# Autodesk Inventor assembly: Assembly1
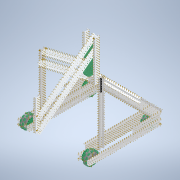
[picture p0: Inventor's stored thumbnail of the model, 180x180]
Saved by Autodesk Inventor 2020 (Build 240168000, 168)
## iProperties
Created: 2019-10-29
Part Number: Assembly1
Document SubType Name: Assembly
Designer: Alex Zaccardelli
Author: Alex Zaccardelli
## Documents named in this file (19)
- D:\DR4BTrayBot\Assembly1.iam
- D:\DR4BTrayBot\SIGBotsCADLibrary-20191023T040826Z-001\SIGBotsCADLibrary\SIGBotsCADLibrary\Structure\C-Channel 5 x 35 (aluminum).ipt
- D:\DR4BTrayBot\SIGBotsCADLibrary-20191023T040826Z-001\SIGBotsCADLibrary\SIGBotsCADLibrary\Structure\C-Channel 3 x 13 (aluminum).ipt
- D:\DR4BTrayBot\SIGBotsCADLibrary-20191023T040826Z-001\SIGBotsCADLibrary\SIGBotsCADLibrary\Structure\C-Channel 2 x 35 (aluminum) New.ipt
- D:\DR4BTrayBot\SIGBotsCADLibrary-20191023T040826Z-001\SIGBotsCADLibrary\SIGBotsCADLibrary\Motion\Spacer 0.50 unit.ipt
- D:\DR4BTrayBot\SIGBotsCADLibrary-20191023T040826Z-001\SIGBotsCADLibrary\SIGBotsCADLibrary\3_25_Omni-Directional_Wheel_276-3526.iam
- D:\DR4BTrayBot\SIGBotsCADLibrary-20191023T040826Z-001\SIGBotsCADLibrary\SIGBotsCADLibrary\Motion\Spacer 0.75 unit.ipt
- D:\DR4BTrayBot\SIGBotsCADLibrary-20191023T040826Z-001\SIGBotsCADLibrary\SIGBotsCADLibrary\Motion\Insert HS Metal.ipt
- D:\DR4BTrayBot\SIGBotsCADLibrary-20191023T040826Z-001\SIGBotsCADLibrary\SIGBotsCADLibrary\Motion\Sprocket HS 18 tooth.ipt
- D:\DR4BTrayBot\SIGBotsCADLibrary-20191023T040826Z-001\SIGBotsCADLibrary\SIGBotsCADLibrary\Structure\C-Channel 3 x 32 (aluminum).ipt
- D:\DR4BTrayBot\SIGBotsCADLibrary-20191023T040826Z-001\SIGBotsCADLibrary\SIGBotsCADLibrary\Structure\C-Channel 2 x 30 (aluminum).ipt
- D:\DR4BTrayBot\SIGBotsCADLibrary-20191023T040826Z-001\SIGBotsCADLibrary\SIGBotsCADLibrary\Motion\Bearing Block.ipt
- D:\DR4BTrayBot\SIGBotsCADLibrary-20191023T040826Z-001\SIGBotsCADLibrary\SIGBotsCADLibrary\Motion\Spacer 0.25 unit.ipt
- D:\DR4BTrayBot\SIGBotsCADLibrary-20191023T040826Z-001\SIGBotsCADLibrary\SIGBotsCADLibrary\Structure\C-Channel 2 x 20 (aluminum).ipt
- D:\DR4BTrayBot\SIGBotsCADLibrary-20191023T040826Z-001\SIGBotsCADLibrary\SIGBotsCADLibrary\Structure\C-Channel 2 x 24 (aluminum).ipt
- D:\DR4BTrayBot\SIGBotsCADLibrary-20191023T040826Z-001\SIGBotsCADLibrary\SIGBotsCADLibrary\Motion\Gear HS 84 tooth.ipt
- D:\DR4BTrayBot\SIGBotsCADLibrary-20191023T040826Z-001\SIGBotsCADLibrary\SIGBotsCADLibrary\Motion\Gear HS 12 tooth.ipt
- D:\DR4BTrayBot\SIGBotsCADLibrary-20191023T040826Z-001\SIGBotsCADLibrary\SIGBotsCADLibrary\Structure\Standoff 1.0 inch.ipt
- D:\DR4BTrayBot\SIGBotsCADLibrary-20191023T040826Z-001\SIGBotsCADLibrary\SIGBotsCADLibrary\Structure\C-Channel 2 x 15 (aluminum).ipt
## Components (56 placed, 18 different names)
1. C-Channel 5 x 35 (aluminum):1 — Mate:1, Mate:2, Mate:3, Mate:42, Mate:48, Mate:49, Mate:50, Mate:54, Mate:55, Mate:56, Mate:88, Mate:89
2. C-Channel 3 x 13 (aluminum):1 — Mate:1, Mate:2, Mate:3, Mate:7, Mate:8, Mate:9, Mate:131
3. C-Channel 2 x 35 (aluminum) New:1 — Mate:7, Mate:8, Mate:9, Mate:39, Mate:40, Mate:41, Mate:131
4. C-Channel 2 x 35 (aluminum) New:2 — Mate:25, Mate:26, Mate:45, Mate:90, Mate:152, Mate:153
5. Spacer 0.50 unit:1 — Mate:41
6. 3_25_Omni-Directional_Wheel_276-3526:1 [sub-assembly]
7. Spacer 0.75 unit:1
8. Insert HS Metal:1
9. Insert HS Metal:2
10. Sprocket HS 18 tooth:1 — Mate:25, Mate:26
11. Spacer 0.50 unit:2
12. 3_25_Omni-Directional_Wheel_276-3526:2 [sub-assembly]
13. Spacer 0.75 unit:2
14. Insert HS Metal:3
15. Insert HS Metal:4
16. Sprocket HS 18 tooth:2 — Mate:39, Mate:40
17. C-Channel 3 x 32 (aluminum):1 — Mate:42, Mate:45, Mate:88, Mate:89, Mate:90, Mate:91
18. C-Channel 3 x 13 (aluminum):2 — Mate:48, Mate:49, Mate:50, Mate:51, Mate:52, Mate:53
19. C-Channel 2 x 35 (aluminum) New:3 — Mate:51, Mate:52, Mate:53, Mate:86
20. C-Channel 3 x 32 (aluminum):2 — Mate:54, Mate:55, Mate:56, Mate:57, Mate:58, Mate:59, Mate:94
21. C-Channel 2 x 35 (aluminum) New:4 — Mate:57, Mate:58, Mate:59, Mate:72, Mate:73, Mate:87, Mate:95, Mate:96
22. Spacer 0.50 unit:3 — Mate:73
23. 3_25_Omni-Directional_Wheel_276-3526:3 [sub-assembly]
24. Spacer 0.75 unit:3
25. Insert HS Metal:5
26. Insert HS Metal:6
27. Sprocket HS 18 tooth:3 — Mate:72
28. Spacer 0.50 unit:4 — Mate:87
29. 3_25_Omni-Directional_Wheel_276-3526:4 [sub-assembly]
30. Spacer 0.75 unit:4
31. Insert HS Metal:7
32. Insert HS Metal:8
33. Sprocket HS 18 tooth:4 — Mate:86
34. C-Channel 2 x 30 (aluminum):1 — Mate:91, Mate:103, Mate:104, Mate:105, Mate:106, Mate:107, Mate:108, Mate:109, Mate:110, Mate:111, Mate:112, Mate:152, Mate:153
35. C-Channel 2 x 30 (aluminum):2 — Mate:94, Mate:95, Mate:96, Mate:97, Mate:98, Mate:99, Mate:100, Mate:101, Mate:102, Mate:113, Mate:114, Mate:115
36. Bearing Block:1 — Mate:97, Mate:98, Mate:99
37. Bearing Block:2 — Mate:100, Mate:101, Mate:102
38. Bearing Block:3 — Mate:103, Mate:104, Mate:105
39. Bearing Block:4 — Mate:106, Mate:107, Mate:108
40. C-Channel 2 x 30 (aluminum):3 — Mate:116, Mate:117, Mate:133, Mate:135, Mate:136, Flush:5, Angle:1, Mate:154
41. Spacer 0.25 unit:1 — Mate:109, Mate:110, Mate:116, Mate:117
42. Spacer 0.25 unit:2 — Mate:111, Mate:112, Mate:143
43. Spacer 0.25 unit:3 — Mate:113
44. Spacer 0.25 unit:4 — Mate:114, Mate:115
45. C-Channel 2 x 20 (aluminum):1 — Mate:133, Mate:135, Mate:137, Mate:138, Mate:139, Mate:144, Mate:145, Mate:146, Mate:147, Mate:148, Flush:7
46. Gear HS 84 tooth:1 — Mate:136, Mate:137, Flush:2, Mate:154
47. Gear HS 84 tooth:2 — Flush:2, Mate:138, Flush:3, Mate:158, Mate:159
48. Gear HS 12 tooth:1 — Mate:139, Flush:3
49. C-Channel 2 x 30 (aluminum):4 — Mate:143, Flush:5, Angle:1, Mate:144
50. C-Channel 2 x 24 (aluminum):1 — Mate:149, Mate:150, Mate:151, Mate:160, Mate:161
51. Standoff 1.0 inch:1 — Mate:145, Mate:146, Mate:149, Mate:151
52. Standoff 1.0 inch:2 — Mate:147, Mate:148, Mate:150
53. C-Channel 2 x 35 (aluminum) New:5 — Mate:158, Mate:159, Flush:6, Angle:2, Mate:164
54. C-Channel 2 x 35 (aluminum) New:6 — Flush:6, Angle:2, Mate:162, Mate:163, Mate:165
55. C-Channel 2 x 20 (aluminum):2 — Flush:7, Mate:160, Mate:161, Mate:162
56. C-Channel 2 x 15 (aluminum):1 — Mate:163, Mate:164, Mate:165
## Relationships (139: Mate 132, Flush 5, Angle 2)
- Mate:1: C-Channel 5 x 35 (aluminum):1 ↔ C-Channel 3 x 13 (aluminum):1
- Mate:2: C-Channel 5 x 35 (aluminum):1 ↔ C-Channel 3 x 13 (aluminum):1
- Mate:3: C-Channel 5 x 35 (aluminum):1 ↔ C-Channel 3 x 13 (aluminum):1
- Mate:7: C-Channel 3 x 13 (aluminum):1 ↔ C-Channel 2 x 35 (aluminum) New:1
- Mate:8: C-Channel 3 x 13 (aluminum):1 ↔ C-Channel 2 x 35 (aluminum) New:1
- Mate:9: C-Channel 3 x 13 (aluminum):1 ↔ C-Channel 2 x 35 (aluminum) New:1
- [Mate]: Spacer 0.75 unit:1 ↔ Sprocket HS 18 tooth:1
- [Mate]: Spacer 0.75 unit:1 ↔ Sprocket HS 18 tooth:1
- [Mate]: 3_25_Omni-Directional_Wheel_276-3526:1 ↔ Insert HS Metal:1
- [Mate]: 3_25_Omni-Directional_Wheel_276-3526:1 ↔ Insert HS Metal:1
- [Mate]: 3_25_Omni-Directional_Wheel_276-3526:1 ↔ Insert HS Metal:1
- [Mate]: 3_25_Omni-Directional_Wheel_276-3526:1 ↔ Insert HS Metal:2
- [Mate]: 3_25_Omni-Directional_Wheel_276-3526:1 ↔ Insert HS Metal:2
- [Mate]: 3_25_Omni-Directional_Wheel_276-3526:1 ↔ Insert HS Metal:2
- [Mate]: Spacer 0.75 unit:1 ↔ Insert HS Metal:1
- [Mate]: Spacer 0.75 unit:1 ↔ Insert HS Metal:1
- [Mate]: Spacer 0.50 unit:1 ↔ Insert HS Metal:2
- [Mate]: Spacer 0.50 unit:1 ↔ Insert HS Metal:2
- Mate:25: C-Channel 2 x 35 (aluminum) New:2 ↔ Sprocket HS 18 tooth:1
- Mate:26: C-Channel 2 x 35 (aluminum) New:2 ↔ Sprocket HS 18 tooth:1
- [Mate]: Spacer 0.75 unit:2 ↔ Sprocket HS 18 tooth:2
- [Mate]: Spacer 0.75 unit:2 ↔ Sprocket HS 18 tooth:2
- [Mate]: 3_25_Omni-Directional_Wheel_276-3526:2 ↔ Insert HS Metal:3
- [Mate]: 3_25_Omni-Directional_Wheel_276-3526:2 ↔ Insert HS Metal:3
- [Mate]: 3_25_Omni-Directional_Wheel_276-3526:2 ↔ Insert HS Metal:3
- [Mate]: 3_25_Omni-Directional_Wheel_276-3526:2 ↔ Insert HS Metal:4
- [Mate]: 3_25_Omni-Directional_Wheel_276-3526:2 ↔ Insert HS Metal:4
- [Mate]: 3_25_Omni-Directional_Wheel_276-3526:2 ↔ Insert HS Metal:4
- [Mate]: Spacer 0.75 unit:2 ↔ Insert HS Metal:3
- [Mate]: Spacer 0.75 unit:2 ↔ Insert HS Metal:3
- [Mate]: Spacer 0.50 unit:2 ↔ Insert HS Metal:4
- [Mate]: Spacer 0.50 unit:2 ↔ Insert HS Metal:4
- Mate:39: C-Channel 2 x 35 (aluminum) New:1 ↔ Sprocket HS 18 tooth:2
- Mate:40: C-Channel 2 x 35 (aluminum) New:1 ↔ Sprocket HS 18 tooth:2
- Mate:41: C-Channel 2 x 35 (aluminum) New:1 ↔ Spacer 0.50 unit:1
- Mate:42: C-Channel 5 x 35 (aluminum):1 ↔ C-Channel 3 x 32 (aluminum):1
- Mate:45: C-Channel 2 x 35 (aluminum) New:2 ↔ C-Channel 3 x 32 (aluminum):1
- Mate:48: C-Channel 5 x 35 (aluminum):1 ↔ C-Channel 3 x 13 (aluminum):2
- Mate:49: C-Channel 5 x 35 (aluminum):1 ↔ C-Channel 3 x 13 (aluminum):2
- Mate:50: C-Channel 5 x 35 (aluminum):1 ↔ C-Channel 3 x 13 (aluminum):2
- Mate:51: C-Channel 3 x 13 (aluminum):2 ↔ C-Channel 2 x 35 (aluminum) New:3
- Mate:52: C-Channel 3 x 13 (aluminum):2 ↔ C-Channel 2 x 35 (aluminum) New:3
- Mate:53: C-Channel 3 x 13 (aluminum):2 ↔ C-Channel 2 x 35 (aluminum) New:3
- Mate:54: C-Channel 5 x 35 (aluminum):1 ↔ C-Channel 3 x 32 (aluminum):2
- Mate:55: C-Channel 5 x 35 (aluminum):1 ↔ C-Channel 3 x 32 (aluminum):2
- Mate:56: C-Channel 5 x 35 (aluminum):1 ↔ C-Channel 3 x 32 (aluminum):2
- Mate:57: C-Channel 3 x 32 (aluminum):2 ↔ C-Channel 2 x 35 (aluminum) New:4
- Mate:58: C-Channel 3 x 32 (aluminum):2 ↔ C-Channel 2 x 35 (aluminum) New:4
- Mate:59: C-Channel 3 x 32 (aluminum):2 ↔ C-Channel 2 x 35 (aluminum) New:4
- [Mate]: Spacer 0.75 unit:3 ↔ Sprocket HS 18 tooth:3
- [Mate]: Spacer 0.75 unit:3 ↔ Sprocket HS 18 tooth:3
- [Mate]: 3_25_Omni-Directional_Wheel_276-3526:3 ↔ Insert HS Metal:5
- [Mate]: 3_25_Omni-Directional_Wheel_276-3526:3 ↔ Insert HS Metal:5
- [Mate]: 3_25_Omni-Directional_Wheel_276-3526:3 ↔ Insert HS Metal:5
- [Mate]: 3_25_Omni-Directional_Wheel_276-3526:3 ↔ Insert HS Metal:6
- [Mate]: 3_25_Omni-Directional_Wheel_276-3526:3 ↔ Insert HS Metal:6
- [Mate]: 3_25_Omni-Directional_Wheel_276-3526:3 ↔ Insert HS Metal:6
- [Mate]: Spacer 0.75 unit:3 ↔ Insert HS Metal:5
- [Mate]: Spacer 0.75 unit:3 ↔ Insert HS Metal:5
- [Mate]: Spacer 0.50 unit:3 ↔ Insert HS Metal:6
- [Mate]: Spacer 0.50 unit:3 ↔ Insert HS Metal:6
- Mate:72: C-Channel 2 x 35 (aluminum) New:4 ↔ Sprocket HS 18 tooth:3
- Mate:73: C-Channel 2 x 35 (aluminum) New:4 ↔ Spacer 0.50 unit:3
- [Mate]: Spacer 0.75 unit:4 ↔ Sprocket HS 18 tooth:4
- [Mate]: Spacer 0.75 unit:4 ↔ Sprocket HS 18 tooth:4
- [Mate]: 3_25_Omni-Directional_Wheel_276-3526:4 ↔ Insert HS Metal:7
- [Mate]: 3_25_Omni-Directional_Wheel_276-3526:4 ↔ Insert HS Metal:7
- [Mate]: 3_25_Omni-Directional_Wheel_276-3526:4 ↔ Insert HS Metal:7
- [Mate]: 3_25_Omni-Directional_Wheel_276-3526:4 ↔ Insert HS Metal:8
- [Mate]: 3_25_Omni-Directional_Wheel_276-3526:4 ↔ Insert HS Metal:8
- [Mate]: 3_25_Omni-Directional_Wheel_276-3526:4 ↔ Insert HS Metal:8
- [Mate]: Spacer 0.75 unit:4 ↔ Insert HS Metal:7
- [Mate]: Spacer 0.75 unit:4 ↔ Insert HS Metal:7
- [Mate]: Spacer 0.50 unit:4 ↔ Insert HS Metal:8
- [Mate]: Spacer 0.50 unit:4 ↔ Insert HS Metal:8
- Mate:86: C-Channel 2 x 35 (aluminum) New:3 ↔ Sprocket HS 18 tooth:4
- Mate:87: C-Channel 2 x 35 (aluminum) New:4 ↔ Spacer 0.50 unit:4
- Mate:88: C-Channel 5 x 35 (aluminum):1 ↔ C-Channel 3 x 32 (aluminum):1
- Mate:89: C-Channel 5 x 35 (aluminum):1 ↔ C-Channel 3 x 32 (aluminum):1
- Mate:90: C-Channel 2 x 35 (aluminum) New:2 ↔ C-Channel 3 x 32 (aluminum):1
- Mate:91: C-Channel 3 x 32 (aluminum):1 ↔ C-Channel 2 x 30 (aluminum):1
- Mate:94: C-Channel 3 x 32 (aluminum):2 ↔ C-Channel 2 x 30 (aluminum):2
- Mate:95: C-Channel 2 x 35 (aluminum) New:4 ↔ C-Channel 2 x 30 (aluminum):2
- Mate:96: C-Channel 2 x 35 (aluminum) New:4 ↔ C-Channel 2 x 30 (aluminum):2
- Mate:97: C-Channel 2 x 30 (aluminum):2 ↔ Bearing Block:1
- Mate:98: C-Channel 2 x 30 (aluminum):2 ↔ Bearing Block:1
- Mate:99: C-Channel 2 x 30 (aluminum):2 ↔ Bearing Block:1
- Mate:100: C-Channel 2 x 30 (aluminum):2 ↔ Bearing Block:2
- Mate:101: C-Channel 2 x 30 (aluminum):2 ↔ Bearing Block:2
- Mate:102: C-Channel 2 x 30 (aluminum):2 ↔ Bearing Block:2
- Mate:103: C-Channel 2 x 30 (aluminum):1 ↔ Bearing Block:3
- Mate:104: C-Channel 2 x 30 (aluminum):1 ↔ Bearing Block:3
- Mate:105: C-Channel 2 x 30 (aluminum):1 ↔ Bearing Block:3
- Mate:106: C-Channel 2 x 30 (aluminum):1 ↔ Bearing Block:4
- Mate:107: C-Channel 2 x 30 (aluminum):1 ↔ Bearing Block:4
- Mate:108: C-Channel 2 x 30 (aluminum):1 ↔ Bearing Block:4
- Mate:109: C-Channel 2 x 30 (aluminum):1 ↔ Spacer 0.25 unit:1
- Mate:110: C-Channel 2 x 30 (aluminum):1 ↔ Spacer 0.25 unit:1
- Mate:111: C-Channel 2 x 30 (aluminum):1 ↔ Spacer 0.25 unit:2
- Mate:112: C-Channel 2 x 30 (aluminum):1 ↔ Spacer 0.25 unit:2
- Mate:113: C-Channel 2 x 30 (aluminum):2 ↔ Spacer 0.25 unit:3
- Mate:114: C-Channel 2 x 30 (aluminum):2 ↔ Spacer 0.25 unit:4
- Mate:115: C-Channel 2 x 30 (aluminum):2 ↔ Spacer 0.25 unit:4
- Mate:116: C-Channel 2 x 30 (aluminum):3 ↔ Spacer 0.25 unit:1
- Mate:117: C-Channel 2 x 30 (aluminum):3 ↔ Spacer 0.25 unit:1
- Mate:131: C-Channel 3 x 13 (aluminum):1 ↔ C-Channel 2 x 35 (aluminum) New:1
- Mate:133: C-Channel 2 x 30 (aluminum):3 ↔ C-Channel 2 x 20 (aluminum):1
- Mate:135: C-Channel 2 x 30 (aluminum):3 ↔ C-Channel 2 x 20 (aluminum):1
- Mate:136 (3.81 mm): C-Channel 2 x 30 (aluminum):3 ↔ Gear HS 84 tooth:1
- Mate:137: C-Channel 2 x 20 (aluminum):1 ↔ Gear HS 84 tooth:1
- Flush:2: Gear HS 84 tooth:1 ↔ Gear HS 84 tooth:2
- Mate:138: C-Channel 2 x 20 (aluminum):1 ↔ Gear HS 84 tooth:2
- Mate:139: C-Channel 2 x 20 (aluminum):1 ↔ Gear HS 12 tooth:1
- Flush:3: Gear HS 84 tooth:2 ↔ Gear HS 12 tooth:1
- Mate:143: Spacer 0.25 unit:2 ↔ C-Channel 2 x 30 (aluminum):4
- Flush:5: C-Channel 2 x 30 (aluminum):3 ↔ C-Channel 2 x 30 (aluminum):4
- Angle:1 (0 deg): C-Channel 2 x 30 (aluminum):3 ↔ C-Channel 2 x 30 (aluminum):4
- Mate:144: C-Channel 2 x 20 (aluminum):1 ↔ C-Channel 2 x 30 (aluminum):4
- Mate:145: C-Channel 2 x 20 (aluminum):1 ↔ Standoff 1.0 inch:1
- Mate:146: C-Channel 2 x 20 (aluminum):1 ↔ Standoff 1.0 inch:1
- Mate:147: C-Channel 2 x 20 (aluminum):1 ↔ Standoff 1.0 inch:2
- Mate:148: C-Channel 2 x 20 (aluminum):1 ↔ Standoff 1.0 inch:2
- Mate:149: C-Channel 2 x 24 (aluminum):1 ↔ Standoff 1.0 inch:1
- Mate:150: C-Channel 2 x 24 (aluminum):1 ↔ Standoff 1.0 inch:2
- Mate:151: C-Channel 2 x 24 (aluminum):1 ↔ Standoff 1.0 inch:1
- Mate:152: C-Channel 2 x 35 (aluminum) New:2 ↔ C-Channel 2 x 30 (aluminum):1
- Mate:153: C-Channel 2 x 35 (aluminum) New:2 ↔ C-Channel 2 x 30 (aluminum):1
- Mate:154: C-Channel 2 x 30 (aluminum):3 ↔ Gear HS 84 tooth:1
- Mate:158 (3.81 mm): Gear HS 84 tooth:2 ↔ C-Channel 2 x 35 (aluminum) New:5
- Mate:159: Gear HS 84 tooth:2 ↔ C-Channel 2 x 35 (aluminum) New:5
- Flush:6: C-Channel 2 x 35 (aluminum) New:5 ↔ C-Channel 2 x 35 (aluminum) New:6
- Angle:2 (0 deg): C-Channel 2 x 35 (aluminum) New:5 ↔ C-Channel 2 x 35 (aluminum) New:6
- Flush:7: C-Channel 2 x 20 (aluminum):1 ↔ C-Channel 2 x 20 (aluminum):2
- Mate:160: C-Channel 2 x 24 (aluminum):1 ↔ C-Channel 2 x 20 (aluminum):2
- Mate:161: C-Channel 2 x 24 (aluminum):1 ↔ C-Channel 2 x 20 (aluminum):2
- Mate:162: C-Channel 2 x 35 (aluminum) New:6 ↔ C-Channel 2 x 20 (aluminum):2
- Mate:163: C-Channel 2 x 35 (aluminum) New:6 ↔ C-Channel 2 x 15 (aluminum):1
- Mate:164: C-Channel 2 x 35 (aluminum) New:5 ↔ C-Channel 2 x 15 (aluminum):1
- Mate:165: C-Channel 2 x 35 (aluminum) New:6 ↔ C-Channel 2 x 15 (aluminum):1
## Named parameters: d35_d185 = 0 mm, d36_d186 = 0 mm, d37_d187 = 0 mm, d38_d188 = 0 mm, d39_d189 = 0 mm, d40_d190 = 0 mm, d41_d191 = 0 mm, d42_d192 = 0 mm, d43_d193 = 0 mm, d44_d194 = 0 mm, d45_d195 = 0 mm, d46_d196 = 0 mm, d68_d185 = 0 mm, d69_d186 = 0 mm, d70_d187 = 0 mm, d71_d188 = 0 mm, d72_d189 = 0 mm, d73_d190 = 0 mm, d74_d191 = 0 mm, d75_d192 = 0 mm, d76_d193 = 0 mm, d77_d194 = 0 mm, d78_d195 = 0 mm, d79_d196 = 0 mm, d82_d185 = 0 mm, d83_d186 = 0 mm, d84_d187 = 0 mm, d85_d188 = 0 mm, d86_d189 = 0 mm, d87_d190 = 0 mm, d88_d191 = 0 mm, d89_d192 = 0 mm, d90_d193 = 0 mm, d91_d194 = 0 mm, d92_d195 = 0 mm, d93_d196 = 0 mm
